# Autodesk Inventor assembly: YaxisNew
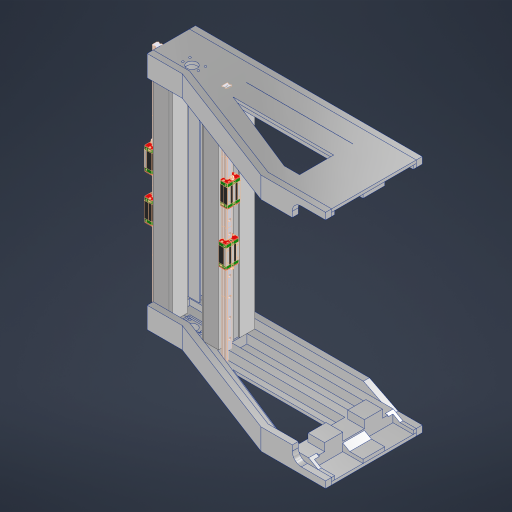
[picture p0: Inventor's stored thumbnail of the model, 512x512]
Saved by Autodesk Inventor 2024 (Build 280153000, 153)
## iProperties
Created: 2023-06-18
Part Number: YaxisNew
Document SubType Name: Assembly
Designer: KirikDK
Mass: 39734.7 g
Surface Area: 33958.7 cm^2
Volume: 15992.4 cm^3
Density: 2.4846 g/cm^3
Author: KirikDK
## Documents named in this file (8)
- C:\Users\KirikDK\Documents\Stanok2023\YaxisNew.iam
- C:\Users\KirikDK\Documents\Stanok2023\YflanecSborka.iam
- C:\Users\KirikDK\Documents\Stanok2023\YaxisUgolok.ipt
- C:\Users\KirikDK\Documents\Stanok2023\BackYflanec.ipt
- C:\Users\KirikDK\Documents\Stanok2023\YKrep.ipt
- C:\Users\KirikDK\Documents\Stanok2023\mgn20_1000.ipt
- C:\Users\KirikDK\Documents\Stanok2023\HGH20_block.ipt
- C:\Users\KirikDK\Documents\Stanok2023\YflanecSborka_MIR.iam
## Components (23 placed, 7 different names)
1. YflanecSborka:1 [sub-assembly] — Mate:1, Flush:1, Flush:2, Mate:2, Mate:3, Flush:3, Mate:4, Flush:4, Flush:5, Mate:5, Mate:6, Flush:6, Mate:12, Mate:15, Mate:16, Mate:21, Mate:39, Mate:41, Mate:44
2. YaxisUgolok:1 — Mate:2, Mate:3, Flush:3, Mate:7, Mate:8, Mate:11, Mate:43, Flush:51
3. YaxisUgolok:2 — Mate:5, Mate:6, Flush:6
4. YaxisUgolok:4 — Mate:4, Flush:4, Flush:5, Mate:17, Mate:18, Flush:49, Mate:38
5. YaxisUgolok:5 — Mate:1, Flush:1, Flush:2, Mate:14, Flush:50, Mate:40
6. BackYflanec:2 — Mate:9, Mate:11, Mate:44
7. YKrep:1 — Mate:7, Mate:8, Mate:9, Mate:12, Mate:13
8. YaxisUgolok:6 — Mate:13, Mate:14, Mate:15, Mate:42
9. YKrep:3 — Mate:16, Mate:17, Mate:18, Mate:19, Mate:20
10. YaxisUgolok:7 — Mate:19, Mate:20, Mate:21
11. mgn20_1000:9
12. mgn20_1000:10 — Flush:50, Mate:41
13. mgn20_1000:11
14. mgn20_1000:12
15. HGH20_block:5
16. HGH20_block:6 — Mate:40
17. mgn20_1000:13 — Flush:49
18. mgn20_1000:14 — Mate:39
19. mgn20_1000:15
20. mgn20_1000:16
21. HGH20_block:7
22. HGH20_block:8 — Mate:38
23. YflanecSborka_MIR:1 [sub-assembly] — Mate:42, Mate:43, Flush:51
## Relationships (62: Mate 33, Flush 29)
- Mate:1: YflanecSborka:1 ↔ YaxisUgolok:5
- Flush:1: YflanecSborka:1 ↔ YaxisUgolok:5
- Flush:2: YflanecSborka:1 ↔ YaxisUgolok:5
- Mate:2: YflanecSborka:1 ↔ YaxisUgolok:1
- Mate:3: YflanecSborka:1 ↔ YaxisUgolok:1
- Flush:3: YflanecSborka:1 ↔ YaxisUgolok:1
- Mate:4: YflanecSborka:1 ↔ YaxisUgolok:4
- Flush:4: YflanecSborka:1 ↔ YaxisUgolok:4
- Flush:5: YflanecSborka:1 ↔ YaxisUgolok:4
- Mate:5: YflanecSborka:1 ↔ YaxisUgolok:2
- Mate:6: YflanecSborka:1 ↔ YaxisUgolok:2
- Flush:6: YflanecSborka:1 ↔ YaxisUgolok:2
- Mate:7: YaxisUgolok:1 ↔ YKrep:1
- Mate:8: YaxisUgolok:1 ↔ YKrep:1
- Mate:9: BackYflanec:2 ↔ YKrep:1
- Mate:11: YaxisUgolok:1 ↔ BackYflanec:2
- Mate:12: YflanecSborka:1 ↔ YKrep:1
- Mate:13: YKrep:1 ↔ YaxisUgolok:6
- Mate:14: YaxisUgolok:5 ↔ YaxisUgolok:6
- Mate:15: YflanecSborka:1 ↔ YaxisUgolok:6
- Mate:16: YflanecSborka:1 ↔ YKrep:3
- Mate:17: YaxisUgolok:4 ↔ YKrep:3
- Mate:18: YaxisUgolok:4 ↔ YKrep:3
- Mate:19: YKrep:3 ↔ YaxisUgolok:7
- Mate:20: YKrep:3 ↔ YaxisUgolok:7
- Mate:21: YflanecSborka:1 ↔ YaxisUgolok:7
- [Mate]: mgn20_1000:9 ↔ mgn20_1000:10
- [Flush]: mgn20_1000:9 ↔ mgn20_1000:10
- [Flush]: mgn20_1000:9 ↔ mgn20_1000:10
- [Mate]: mgn20_1000:11 ↔ mgn20_1000:12
- [Flush]: mgn20_1000:11 ↔ mgn20_1000:12
- [Flush]: mgn20_1000:11 ↔ mgn20_1000:12
- [Mate]: mgn20_1000:9 ↔ mgn20_1000:12
- [Flush]: mgn20_1000:9 ↔ mgn20_1000:12
- [Flush]: mgn20_1000:9 ↔ mgn20_1000:12
- [Flush]: mgn20_1000:11 ↔ HGH20_block:5
- [Flush]: mgn20_1000:11 ↔ HGH20_block:5
- [Flush]: mgn20_1000:9 ↔ HGH20_block:6
- [Flush]: mgn20_1000:9 ↔ HGH20_block:6
- [Mate]: mgn20_1000:13 ↔ mgn20_1000:14
- [Flush]: mgn20_1000:13 ↔ mgn20_1000:14
- [Flush]: mgn20_1000:13 ↔ mgn20_1000:14
- [Mate]: mgn20_1000:15 ↔ mgn20_1000:16
- [Flush]: mgn20_1000:15 ↔ mgn20_1000:16
- [Flush]: mgn20_1000:15 ↔ mgn20_1000:16
- [Mate]: mgn20_1000:13 ↔ mgn20_1000:16
- [Flush]: mgn20_1000:13 ↔ mgn20_1000:16
- [Flush]: mgn20_1000:13 ↔ mgn20_1000:16
- [Flush]: mgn20_1000:16 ↔ HGH20_block:8
- [Flush]: mgn20_1000:13 ↔ HGH20_block:8
- [Flush]: mgn20_1000:16 ↔ HGH20_block:7
- [Flush]: mgn20_1000:16 ↔ HGH20_block:7
- Flush:49: YaxisUgolok:4 ↔ mgn20_1000:13
- Mate:38: YaxisUgolok:4 ↔ HGH20_block:8
- Mate:39: YflanecSborka:1 ↔ mgn20_1000:14
- Flush:50: YaxisUgolok:5 ↔ mgn20_1000:10
- Mate:40: YaxisUgolok:5 ↔ HGH20_block:6
- Mate:41: YflanecSborka:1 ↔ mgn20_1000:10
- Mate:42: YaxisUgolok:6 ↔ YflanecSborka_MIR:1
- Mate:43: YaxisUgolok:1 ↔ YflanecSborka_MIR:1
- Flush:51: YaxisUgolok:1 ↔ YflanecSborka_MIR:1
- Mate:44: YflanecSborka:1 ↔ BackYflanec:2
## Named parameters: d68_d45_d38 = 0 mm, d69_d46_d39_d38 = 0 mm, d70_d47_d40_d36 = 0 mm, d71_d48_d41_d37 = 0 mm, d72_d49_d42 = 0 mm, d73_d50_d43 = 0 mm, d74_d51_d44 = 0 mm, d75_d52_d36 = 0 mm, d76_d53_d37 = 0 mm, d77_d60 = 0 mm, d78_d61 = 0 mm, d79_d62 = 0 mm, d80_d63 = 0 mm, d81_d38 = 0 mm, d82_d39_d38 = 0 mm, d83_d40_d36 = 0 mm, d84_d41_d37 = 0 mm, d85_d42 = 0 mm, d86_d43 = 0 mm, d87_d44 = 0 mm, d88_d36 = 0 mm, d89_d37 = 0 mm, d90_d65 = 0 mm, d91_d66 = 0 mm, d92_d67 = 0 mm, d93_d64 = 0 mm
